# Autodesk Inventor assembly: Сборка
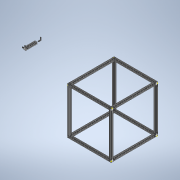
[picture p0: Inventor's stored thumbnail of the model, 180x180]
Saved by Autodesk Inventor 2020 (Build 240168000, 168)
## iProperties
Created: 2019-09-20
Part Number: Сборка
Document SubType Name: Assembly
Designer: Михаил
Author: Михаил
## Documents named in this file (6)
- D:\MyWorks\GrowBox_v2\3D_body\Сборка.iam
- D:\MyWorks\GrowBox_v2\3D_body\Профиль_аллюминиевый.ipt
- D:\MyWorks\GrowBox_v2\3D_body\L-connector2020.ipt
- D:\MyWorks\GrowBox_v2\3D_body\new_Lconnector20202065.ipt
- D:\MyWorks\GrowBox_v2\3D_body\new_profile2020OB-2020.ipt
- D:\MyWorks\GrowBox_v2\3D_body\2004.ipt
## Components (23 placed, 5 different names)
1. Профиль_алюминиевый:1 — Совмещение:1, Заподлицо:1, Совмещение:2, Совмещение:3, Заподлицо:2, Заподлицо:3, Совмещение:4, Совмещение:5, Заподлицо:7, Обкатка:1, Заподлицо:36, Заподлицо:37
2. L-connector2020:1 — Совмещение:3, Заподлицо:2, Заподлицо:3, Заподлицо:4, Заподлицо:5, Заподлицо:6
3. Профиль_алюминиевый:2 — Совмещение:4, Заподлицо:4, Заподлицо:5, Совмещение:11, Заподлицо:16, Заподлицо:17
4. Профиль_алюминиевый:3 — Совмещение:5, Заподлицо:6, Заподлицо:7, Совмещение:6, Заподлицо:8, Заподлицо:9, Заподлицо:21
5. L-connector2020:2 — Совмещение:6, Заподлицо:8, Заподлицо:9, Совмещение:7, Заподлицо:10, Заподлицо:11, Совмещение:14
6. Профиль_алюминиевый:4 — Совмещение:7, Заподлицо:10, Заподлицо:11, Совмещение:8, Заподлицо:12, Заподлицо:13, Заподлицо:20, Заподлицо:22
7. L-connector2020:3 — Совмещение:8, Заподлицо:12, Заподлицо:13, Совмещение:9, Заподлицо:14, Заподлицо:15, Совмещение:13
8. Профиль_алюминиевый:5 — Совмещение:9, Заподлицо:14, Заподлицо:15, Совмещение:10, Заподлицо:18, Заподлицо:19
9. L-connector2020:4 — Совмещение:10, Совмещение:11, Заподлицо:16, Совмещение:12
10. Профиль_алюминиевый:6 — Совмещение:12, Заподлицо:17, Заподлицо:18, Заподлицо:38
11. Профиль_алюминиевый:7 — Совмещение:13, Заподлицо:19, Заподлицо:20
12. Профиль_алюминиевый:8 — Совмещение:14, Заподлицо:21, Заподлицо:22
13. L-connector2020:5 — Совмещение:21, Совмещение:22, Заподлицо:35, Заподлицо:38, Заподлицо:39, Заподлицо:40
14. Профиль_алюминиевый:9 — Совмещение:21, Заподлицо:39
15. Профиль_алюминиевый:10 — Совмещение:22, Заподлицо:35, Заподлицо:40
16. L-connector2020:6
17. Профиль_алюминиевый:11
18. L-connector2020:7
19. Профиль_алюминиевый:12
20. L-connector2020:8 — Обкатка:1, Заподлицо:36, Заподлицо:37
21. new_Lconnector20202065:1 — Совмещение:23, Заподлицо:41, Заподлицо:42
22. new_profile2020OB-2020:1 — Совмещение:23, Заподлицо:41, Заподлицо:42
23. 2004:1
## Relationships (66: Flush 42, Mate 23, Transitional 1)
- Совмещение:1 [Mate]: Профиль_алюминиевый:1
- Заподлицо:1 [Flush]: Профиль_алюминиевый:1
- Совмещение:2 [Mate]: Профиль_алюминиевый:1
- Совмещение:3 [Mate]: Профиль_алюминиевый:1 ↔ L-connector2020:1
- Заподлицо:2 [Flush]: Профиль_алюминиевый:1 ↔ L-connector2020:1
- Заподлицо:3 [Flush]: Профиль_алюминиевый:1 ↔ L-connector2020:1
- Совмещение:4 [Mate]: Профиль_алюминиевый:1 ↔ Профиль_алюминиевый:2
- Заподлицо:4 [Flush]: L-connector2020:1 ↔ Профиль_алюминиевый:2
- Заподлицо:5 [Flush]: L-connector2020:1 ↔ Профиль_алюминиевый:2
- Совмещение:5 [Mate]: Профиль_алюминиевый:1 ↔ Профиль_алюминиевый:3
- Заподлицо:6 [Flush]: L-connector2020:1 ↔ Профиль_алюминиевый:3
- Заподлицо:7 [Flush]: Профиль_алюминиевый:1 ↔ Профиль_алюминиевый:3
- Совмещение:6 [Mate]: Профиль_алюминиевый:3 ↔ L-connector2020:2
- Заподлицо:8 [Flush]: Профиль_алюминиевый:3 ↔ L-connector2020:2
- Заподлицо:9 [Flush]: Профиль_алюминиевый:3 ↔ L-connector2020:2
- Совмещение:7 [Mate]: L-connector2020:2 ↔ Профиль_алюминиевый:4
- Заподлицо:10 [Flush]: L-connector2020:2 ↔ Профиль_алюминиевый:4
- Заподлицо:11 [Flush]: L-connector2020:2 ↔ Профиль_алюминиевый:4
- Совмещение:8 [Mate]: Профиль_алюминиевый:4 ↔ L-connector2020:3
- Заподлицо:12 [Flush]: Профиль_алюминиевый:4 ↔ L-connector2020:3
- Заподлицо:13 [Flush]: Профиль_алюминиевый:4 ↔ L-connector2020:3
- Совмещение:9 [Mate]: L-connector2020:3 ↔ Профиль_алюминиевый:5
- Заподлицо:14 [Flush]: L-connector2020:3 ↔ Профиль_алюминиевый:5
- Заподлицо:15 [Flush]: L-connector2020:3 ↔ Профиль_алюминиевый:5
- Совмещение:10 [Mate]: Профиль_алюминиевый:5 ↔ L-connector2020:4
- Совмещение:11 [Mate]: Профиль_алюминиевый:2 ↔ L-connector2020:4
- Заподлицо:16 [Flush]: Профиль_алюминиевый:2 ↔ L-connector2020:4
- Совмещение:12 [Mate]: L-connector2020:4 ↔ Профиль_алюминиевый:6
- Заподлицо:17 [Flush]: Профиль_алюминиевый:2 ↔ Профиль_алюминиевый:6
- Заподлицо:18 [Flush]: Профиль_алюминиевый:5 ↔ Профиль_алюминиевый:6
- Совмещение:13 [Mate]: L-connector2020:3 ↔ Профиль_алюминиевый:7
- Заподлицо:19 [Flush]: Профиль_алюминиевый:5 ↔ Профиль_алюминиевый:7
- Заподлицо:20 [Flush]: Профиль_алюминиевый:4 ↔ Профиль_алюминиевый:7
- Совмещение:14 [Mate]: L-connector2020:2 ↔ Профиль_алюминиевый:8
- Заподлицо:21 [Flush]: Профиль_алюминиевый:3 ↔ Профиль_алюминиевый:8
- Заподлицо:22 [Flush]: Профиль_алюминиевый:4 ↔ Профиль_алюминиевый:8
- [Flush]: L-connector2020:5 ↔ Профиль_алюминиевый:9
- [Flush]: L-connector2020:5 ↔ Профиль_алюминиевый:9
- [Flush]: L-connector2020:5 ↔ Профиль_алюминиевый:10
- [Mate]: Профиль_алюминиевый:10 ↔ L-connector2020:6
- [Flush]: Профиль_алюминиевый:10 ↔ L-connector2020:6
- [Flush]: Профиль_алюминиевый:10 ↔ L-connector2020:6
- [Mate]: L-connector2020:6 ↔ Профиль_алюминиевый:11
- [Flush]: L-connector2020:6 ↔ Профиль_алюминиевый:11
- [Flush]: L-connector2020:6 ↔ Профиль_алюминиевый:11
- [Mate]: Профиль_алюминиевый:11 ↔ L-connector2020:7
- [Flush]: Профиль_алюминиевый:11 ↔ L-connector2020:7
- [Flush]: Профиль_алюминиевый:11 ↔ L-connector2020:7
- [Mate]: L-connector2020:7 ↔ Профиль_алюминиевый:12
- [Flush]: L-connector2020:7 ↔ Профиль_алюминиевый:12
- [Flush]: L-connector2020:7 ↔ Профиль_алюминиевый:12
- [Mate]: Профиль_алюминиевый:12 ↔ L-connector2020:8
- [Mate]: Профиль_алюминиевый:9 ↔ L-connector2020:8
- [Flush]: Профиль_алюминиевый:9 ↔ L-connector2020:8
- Совмещение:21 [Mate]: L-connector2020:5 ↔ Профиль_алюминиевый:9
- Совмещение:22 [Mate]: L-connector2020:5 ↔ Профиль_алюминиевый:10
- Заподлицо:35 [Flush]: L-connector2020:5 ↔ Профиль_алюминиевый:10
- Обкатка:1 [Transitional]: Профиль_алюминиевый:1 ↔ L-connector2020:8
- Заподлицо:36 [Flush]: Профиль_алюминиевый:1 ↔ L-connector2020:8
- Заподлицо:37 [Flush]: Профиль_алюминиевый:1 ↔ L-connector2020:8
- Заподлицо:38 [Flush]: Профиль_алюминиевый:6 ↔ L-connector2020:5
- Заподлицо:39 [Flush]: L-connector2020:5 ↔ Профиль_алюминиевый:9
- Заподлицо:40 [Flush]: L-connector2020:5 ↔ Профиль_алюминиевый:10
- Совмещение:23 [Mate]: new_Lconnector20202065:1 ↔ new_profile2020OB-2020:1
- Заподлицо:41 [Flush]: new_Lconnector20202065:1 ↔ new_profile2020OB-2020:1
- Заподлицо:42 [Flush]: new_Lconnector20202065:1 ↔ new_profile2020OB-2020:1
## Named parameters: d112_d102 = 0 mm, d113_d93 = 0 mm, d114_d94 = 0 mm, d115_d95 = 0 mm, d116_d96 = 0 mm, d117_d97 = 0 mm, d118_d98 = 0 mm, d119_d99 = 0 mm, d120_d100 = 0 mm, d121_d101 = 0 mm, d122_d84 = 0 mm, d123_d86 = 0 mm, d124_d88 = 0 mm, d125_d89 = 0 mm, d126_d90 = 0 mm, d127_d91 = 0 mm, d128_d92 = 0 mm, d129_d83 = 0 mm
